# Autodesk Inventor assembly: box assembly
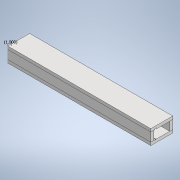
[picture p0: Inventor's stored thumbnail of the model, 180x180]
Saved by Autodesk Inventor 2021 (Build 250183000, 183)
## iProperties
Created: 2021-07-05
Part Number: box assembly
Document SubType Name: Assembly
Designer: newic
Author: newic
## Documents named in this file (5)
- C:\Users\newic\OneDrive\Desktop\ODM\box\box assembly.iam
- C:\Users\newic\OneDrive\Desktop\ODM\box\small bourd.ipt
- C:\Users\newic\OneDrive\Desktop\ODM\box\frount plate.ipt
- C:\Users\newic\OneDrive\Desktop\ODM\box\big bourd bot.ipt
- C:\Users\newic\OneDrive\Desktop\ODM\box\big bourd top.ipt
## Components (5 placed, 4 different names)
1. small bourd:1 — Flush:6, Mate:1, Mate:3, Flush:8
2. small bourd:2 — Flush:7
3. frount plate:1 — Flush:6, Mate:2, Mate:4
4. big bourd bot:1 — Mate:3, Mate:4, Flush:8
5. big bourd top:1 — Mate:1, Mate:2, Flush:7
## Relationships (7: Mate 4, Flush 3)
- Flush:6: small bourd:1 ↔ frount plate:1
- Mate:1: small bourd:1 ↔ big bourd top:1
- Mate:2: frount plate:1 ↔ big bourd top:1
- Flush:7: small bourd:2 ↔ big bourd top:1
- Mate:3: small bourd:1 ↔ big bourd bot:1
- Mate:4: frount plate:1 ↔ big bourd bot:1
- Flush:8: small bourd:1 ↔ big bourd bot:1
